# Autodesk Inventor assembly: forward brace frame
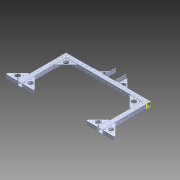
[picture p0: Inventor's stored thumbnail of the model, 180x180]
Saved by Autodesk Inventor 2014 SP1 (Build 180222100, 222)
## iProperties
Created: 2014-01-06
Part Number: forward brace frame
Document SubType Name: Assembly
Designer: Arpan
Author: Arpan
## Documents named in this file (4)
- C:\Users\Arpan\Documents\GitHub\2014buildCAD\Shooter\forward brace frame.iam
- C:\Users\Arpan\Documents\GitHub\2014buildCAD\Shooter\Vex Pro 1x1 rectangular tubing 11 in length.ipt
- C:\Users\Arpan\Documents\GitHub\2014buildCAD\Shooter\Vex Pro Corner Gusset.ipt
- C:\Users\Arpan\Documents\GitHub\2014buildCAD\Shooter\Vex Pro 1x1 rectangular tubing 21 in length.ipt
## Components (11 placed, 3 different names)
1. Vex Pro 1x1 rectangular tubing 11 in length:1 — Mate:1, Flush:1, Flush:2, Mate:2, Mate:3, Mate:4, Mate:8, Mate:9, Mate:10, Mate:11, Mate:12, Mate:13, Flush:3, Flush:4
2. Vex Pro 1x1 rectangular tubing 11 in length:2 — Mate:1, Flush:1, Flush:2, Mate:5, Mate:6, Mate:7, Mate:14, Mate:15, Mate:16, Mate:17, Mate:18, Mate:19
3. Vex Pro Corner Gusset:1 — Mate:11, Mate:12, Mate:13
4. Vex Pro Corner Gusset:2 — Mate:8, Mate:9, Mate:10
5. Vex Pro Corner Gusset:3 — Mate:17, Mate:18, Mate:19
6. Vex Pro Corner Gusset:4 — Mate:14, Mate:15, Mate:16
7. Vex Pro Corner Gusset:5 — Mate:5, Mate:6, Mate:7
8. Vex Pro Corner Gusset:6 — Mate:2, Mate:3, Mate:4, Mate:20
9. Vex Pro 1x1 rectangular tubing 21 in length:1 — Mate:20, Flush:3, Flush:4, Mate:21, Flush:5, Mate:22, Flush:6, Mate:23
10. Vex Pro Corner Gusset:7 — Mate:21, Flush:5, Mate:23
11. Vex Pro Corner Gusset:8 — Mate:22, Flush:6
## Relationships (29: Mate 23, Flush 6)
- Mate:1 (482.6 mm): Vex Pro 1x1 rectangular tubing 11 in length:1 ↔ Vex Pro 1x1 rectangular tubing 11 in length:2
- Flush:1: Vex Pro 1x1 rectangular tubing 11 in length:1 ↔ Vex Pro 1x1 rectangular tubing 11 in length:2
- Flush:2: Vex Pro 1x1 rectangular tubing 11 in length:1 ↔ Vex Pro 1x1 rectangular tubing 11 in length:2
- Mate:2: Vex Pro 1x1 rectangular tubing 11 in length:1 ↔ Vex Pro Corner Gusset:6
- Mate:3: Vex Pro 1x1 rectangular tubing 11 in length:1 ↔ Vex Pro Corner Gusset:6
- Mate:4: Vex Pro 1x1 rectangular tubing 11 in length:1 ↔ Vex Pro Corner Gusset:6
- Mate:5: Vex Pro 1x1 rectangular tubing 11 in length:2 ↔ Vex Pro Corner Gusset:5
- Mate:6: Vex Pro 1x1 rectangular tubing 11 in length:2 ↔ Vex Pro Corner Gusset:5
- Mate:7: Vex Pro 1x1 rectangular tubing 11 in length:2 ↔ Vex Pro Corner Gusset:5
- Mate:8: Vex Pro 1x1 rectangular tubing 11 in length:1 ↔ Vex Pro Corner Gusset:2
- Mate:9: Vex Pro 1x1 rectangular tubing 11 in length:1 ↔ Vex Pro Corner Gusset:2
- Mate:10: Vex Pro 1x1 rectangular tubing 11 in length:1 ↔ Vex Pro Corner Gusset:2
- Mate:11: Vex Pro 1x1 rectangular tubing 11 in length:1 ↔ Vex Pro Corner Gusset:1
- Mate:12: Vex Pro 1x1 rectangular tubing 11 in length:1 ↔ Vex Pro Corner Gusset:1
- Mate:13: Vex Pro 1x1 rectangular tubing 11 in length:1 ↔ Vex Pro Corner Gusset:1
- Mate:14: Vex Pro 1x1 rectangular tubing 11 in length:2 ↔ Vex Pro Corner Gusset:4
- Mate:15: Vex Pro 1x1 rectangular tubing 11 in length:2 ↔ Vex Pro Corner Gusset:4
- Mate:16: Vex Pro 1x1 rectangular tubing 11 in length:2 ↔ Vex Pro Corner Gusset:4
- Mate:17: Vex Pro 1x1 rectangular tubing 11 in length:2 ↔ Vex Pro Corner Gusset:3
- Mate:18: Vex Pro 1x1 rectangular tubing 11 in length:2 ↔ Vex Pro Corner Gusset:3
- Mate:19: Vex Pro 1x1 rectangular tubing 11 in length:2 ↔ Vex Pro Corner Gusset:3
- Mate:20: Vex Pro Corner Gusset:6 ↔ Vex Pro 1x1 rectangular tubing 21 in length:1
- Flush:3: Vex Pro 1x1 rectangular tubing 11 in length:1 ↔ Vex Pro 1x1 rectangular tubing 21 in length:1
- Flush:4: Vex Pro 1x1 rectangular tubing 11 in length:1 ↔ Vex Pro 1x1 rectangular tubing 21 in length:1
- Mate:21: Vex Pro 1x1 rectangular tubing 21 in length:1 ↔ Vex Pro Corner Gusset:7
- Flush:5: Vex Pro 1x1 rectangular tubing 21 in length:1 ↔ Vex Pro Corner Gusset:7
- Mate:22: Vex Pro 1x1 rectangular tubing 21 in length:1 ↔ Vex Pro Corner Gusset:8
- Flush:6: Vex Pro 1x1 rectangular tubing 21 in length:1 ↔ Vex Pro Corner Gusset:8
- Mate:23: Vex Pro 1x1 rectangular tubing 21 in length:1 ↔ Vex Pro Corner Gusset:7
